# Autodesk Inventor assembly: SumoAssembly
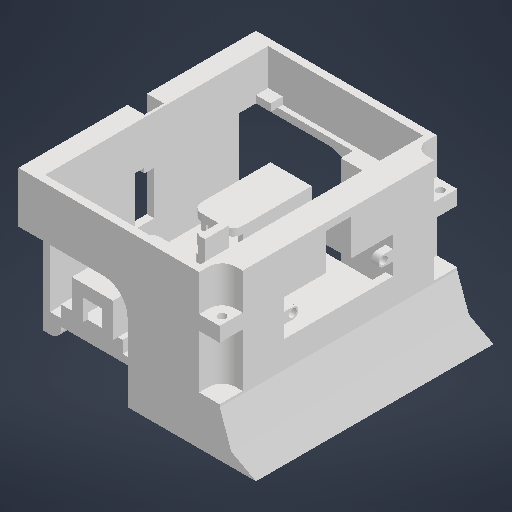
[picture p0: Inventor's stored thumbnail of the model, 512x512]
Saved by Autodesk Inventor 2026 (Build 300175000, 175)
## iProperties
Created: 2026-05-16
Part Number: SumoAssembly
Document SubType Name: Assembly
Designer: Patryk Lombardo
Author: Patryk Lombardo
## Documents named in this file (5)
- C:\Users\Patryk Lombardo\Desktop\sumo\SumoAssembly.iam
- C:\Users\Patryk Lombardo\Desktop\sumo\BodyTop.ipt
- C:\Users\Patryk Lombardo\Desktop\sumo\MotorA.ipt
- C:\Users\Patryk Lombardo\Desktop\sumo\MotorB.ipt
- C:\Users\Patryk Lombardo\Desktop\sumo\BodyBottom.ipt
## Components (4 placed, 4 different names)
1. BodyTop:1 — Zestawiające:1, Zestawiające:2
2. MotorA:1 — Zestawiające:3, Zestawiające:4
3. MotorB:1 — Zestawiające:5, Zestawiające:6
4. BodyBottom:1 — Zestawiające:1, Zestawiające:2, Zestawiające:3, Zestawiające:4, Zestawiające:5, Zestawiające:6
## Relationships (6: Mate 6)
- Zestawiające:1 [Mate]: BodyTop:1 ↔ BodyBottom:1
- Zestawiające:2 [Mate]: BodyTop:1 ↔ BodyBottom:1
- Zestawiające:3 [Mate]: MotorA:1 ↔ BodyBottom:1
- Zestawiające:4 [Mate]: MotorA:1 ↔ BodyBottom:1
- Zestawiające:5 [Mate]: MotorB:1 ↔ BodyBottom:1
- Zestawiające:6 [Mate]: MotorB:1 ↔ BodyBottom:1
